# Autodesk Inventor assembly: obj5
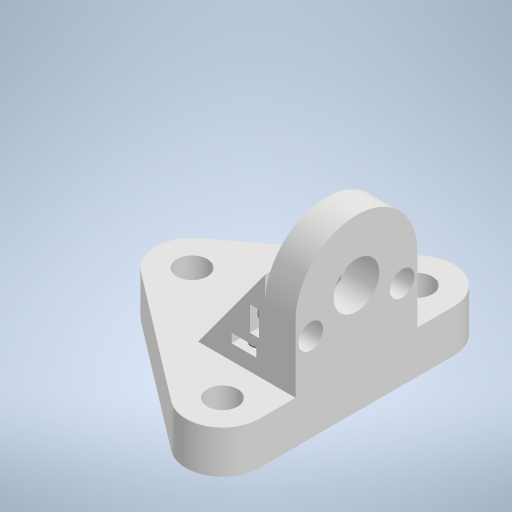
[picture p0: Inventor's stored thumbnail of the model, 512x512]
Saved by Autodesk Inventor 2023.2 (Build 272271030, 271C)
## iProperties
Created: 2023-02-25
Part Number: obj5
Document SubType Name: Assembly
Designer: Cris Pat
Author: Cris Pat
## Documents named in this file (6)
- C:\Users\Cris Pat\Desktop\U\Semestre 9\disenio e innovacion\CAD\obj5.iam
- C:\Users\Cris Pat\Desktop\U\Semestre 9\disenio e innovacion\CAD\arco_obj4.ipt
- C:\Users\Cris Pat\Desktop\U\Semestre 9\disenio e innovacion\CAD\base_obj4.ipt
- C:\Users\Cris Pat\Desktop\U\Semestre 9\disenio e innovacion\CAD\ligamento_obj4.ipt
- C:\Users\Cris Pat\Documents\Inventor\Content Center Files\R2023\en-US\DIN 84\DIN 84 - M5 x 8.ipt
- C:\Users\Cris Pat\Documents\Inventor\Content Center Files\R2023\en-US\DIN 84\DIN 84 - M5 x 20.ipt
## Components (8 placed, 5 different names)
1. arco_obj4:1 — Rigid:1, Rigid:2, Rotational:2, Rotational:3
2. base_obj4:1 — Rotational:1, Rotational:4, Rotational:5
3. ligamento_obj4:1 — Rigid:1
4. ligamento_obj4:2 — Rigid:2, Rotational:1
5. DIN 84 - replaced by DIN EN ISO 1207 M5 x 8:1 — Rotational:2
6. DIN 84 - replaced by DIN EN ISO 1207 M5 x 8:2 — Rotational:3
7. DIN 84 - replaced by DIN EN ISO 1207 M5 x 20:1 — Rotational:4
8. DIN 84 - replaced by DIN EN ISO 1207 M5 x 20:2 — Rotational:5
## Relationships (7: RevoluteJoint 5, WeldJoint 2)
- Rigid:1 [WeldJoint]: arco_obj4:1 ↔ ligamento_obj4:1
- Rigid:2 [WeldJoint]: arco_obj4:1 ↔ ligamento_obj4:2
- Rotational:1 [RevoluteJoint]: base_obj4:1 ↔ ligamento_obj4:2
- Rotational:2 [RevoluteJoint]: arco_obj4:1 ↔ DIN 84 - replaced by DIN EN ISO 1207 M5 x 8:1
- Rotational:3 [RevoluteJoint]: arco_obj4:1 ↔ DIN 84 - replaced by DIN EN ISO 1207 M5 x 8:2
- Rotational:4 [RevoluteJoint]: base_obj4:1 ↔ DIN 84 - replaced by DIN EN ISO 1207 M5 x 20:1
- Rotational:5 [RevoluteJoint]: base_obj4:1 ↔ DIN 84 - replaced by DIN EN ISO 1207 M5 x 20:2
